# Autodesk Inventor assembly: ActiveClimb-ver2-1111-2020
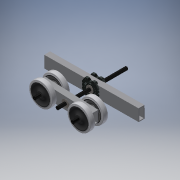
[picture p0: Inventor's stored thumbnail of the model, 180x180]
Saved by Autodesk Inventor 2018 (Build 220112000, 112)
## iProperties
Created: 2020-01-27
Part Number: ActiveClimb-ver2-1111-2020
Document SubType Name: Assembly
Designer: JMHal
Author: JMHal
## Documents named in this file (10)
- G:\PHRC Design Team\GrabCAD\Power Hawks CAD\2020 Infinite Recharge\Active Climb\Assemblies\ActiveClimb-ver2-1111-2020.iam
- G:\PHRC Design Team\GrabCAD\Power Hawks CAD\2020 Infinite Recharge\Active Climb\Parts\AluminumBar-1111-2020.ipt
- G:\PHRC Design Team\GrabCAD\Power Hawks CAD\Resources\VEXpro Resources\Bearings\0.5inHexFlangedBearing(1.125inx0.313in)-1111-2016.ipt
- F:\GrabCad\Resources\VEXpro Resources\Shafts\0.5inThunderHexShaft(8)-1111-2016.ipt
- G:\PHRC Design Team\GrabCAD\Power Hawks CAD\Resources\VEXpro Resources\Wheels\4 inch\4inColsonPerformaWheel-1111-2017.ipt
- G:\PHRC Design Team\GrabCAD\Power Hawks CAD\2020 Infinite Recharge\Active Climb\Parts\2x1 16in Aluminum-ver1-1111-2020.ipt
- G:\PHRC Design Team\GrabCAD\Power Hawks CAD\Resources\VEXpro Resources\Versa Motion\VersaBlockKit-1111-2016.ipt
- G:\PHRC Design Team\GrabCAD\Power Hawks CAD\2020 Infinite Recharge\Active Climb\Parts\12in Hex Shaft-ver1-1111-2020.iam
- G:\PHRC Design Team\GrabCAD\Power Hawks CAD\Resources\VEXpro Resources\Shafts\0.5inThunderHexShaft(8in(modified))-1111-2016.ipt
- G:\PHRC Design Team\GrabCAD\Power Hawks CAD\Resources\VEXpro Resources\Shafts\0.5inThunderHexShaft(5in(modified))-1111-2016.ipt
## Components (22 placed, 9 different names)
1. AluminumBar-1111-2020:1 — Cylindrical:1, Mate:1, Cylindrical:2, Mate:2, Cylindrical:3, Mate:3, Cylindrical:4, Mate:4, Cylindrical:5, Mate:5, Cylindrical:6, Mate:6
2. 0.5inThunderHexShaft(8)-1111-2016:1 — Cylindrical:16, Cylindrical:17, Flush:1, Cylindrical:21
3. 0.5inThunderHexShaft(8)-1111-2016:3 — Cylindrical:19, Flush:3, Cylindrical:20, Cylindrical:22
4. 4inColsonPerformaWheel-1111-2017:1 — Cylindrical:16, Mate:7, Cylindrical:30
5. 4inColsonPerformaWheel-1111-2017:2 — Cylindrical:20, Mate:8, Cylindrical:32
6. 4inColsonPerformaWheel-1111-2017:3 — Cylindrical:21, Mate:9, Cylindrical:34
7. 4inColsonPerformaWheel-1111-2017:4 — Cylindrical:22, Mate:10, Cylindrical:33
8. 2x1 16in Aluminum-ver1-1111-2020:1 — Mate:11, Mate:12, Angle:2, Mate:13, Mate:14, Angle:3
9. VersaBlockKit-1111-2016:1 — Mate:11, Mate:12, Angle:2, Cylindrical:24, Mate:15
10. VersaBlockKit-1111-2016:2 — Mate:13, Mate:14, Angle:3, Cylindrical:25, Mate:16
11. 0.5inHexFlangedBearing(1.125inx0.313in)-1111-2016:7 — Cylindrical:24, Mate:15, Cylindrical:27, Cylindrical:35, Flush:7, Mate:17
12. 0.5inHexFlangedBearing(1.125inx0.313in)-1111-2016:8 — Cylindrical:25, Mate:16
13. 12in Hex Shaft-ver1-1111-2020:1 [sub-assembly] — Cylindrical:26, Cylindrical:27
14. 0.5inThunderHexShaft(5in(modified))-1111-2016:1 — Cylindrical:29, Flush:5, Cylindrical:30, Cylindrical:34
15. 0.5inThunderHexShaft(5in(modified))-1111-2016:2 — Cylindrical:31, Flush:6, Cylindrical:32, Cylindrical:33
16. 0.5inThunderHexShaft(8in(modified))-1111-2016:2 — Cylindrical:35, Flush:7, Cylindrical:36
17. 0.5inHexFlangedBearing(1.125inx0.313in)-1111-2016:2 — Cylindrical:2, Mate:2, Cylindrical:26, Cylindrical:36
18. 0.5inHexFlangedBearing(1.125inx0.313in)-1111-2016:1 — Cylindrical:1, Mate:1, Cylindrical:17, Flush:1, Mate:7, Cylindrical:29, Flush:5
19. 0.5inHexFlangedBearing(1.125inx0.313in)-1111-2016:3 — Cylindrical:3, Mate:3, Cylindrical:19, Flush:3, Mate:8, Cylindrical:31, Flush:6
20. 0.5inHexFlangedBearing(1.125inx0.313in)-1111-2016:4 — Cylindrical:4, Mate:4, Mate:10
21. 0.5inHexFlangedBearing(1.125inx0.313in)-1111-2016:5 — Cylindrical:5, Mate:5, Mate:17
22. 0.5inHexFlangedBearing(1.125inx0.313in)-1111-2016:6 — Cylindrical:6, Mate:6, Mate:9
## Relationships (48: CylindricalJoint 24, Mate 17, Flush 5, Angle 2)
- Cylindrical:1: AluminumBar-1111-2020:1 ↔ 0.5inHexFlangedBearing(1.125inx0.313in)-1111-2016:1
- Mate:1: AluminumBar-1111-2020:1 ↔ 0.5inHexFlangedBearing(1.125inx0.313in)-1111-2016:1
- Cylindrical:2: AluminumBar-1111-2020:1 ↔ 0.5inHexFlangedBearing(1.125inx0.313in)-1111-2016:2
- Mate:2: AluminumBar-1111-2020:1 ↔ 0.5inHexFlangedBearing(1.125inx0.313in)-1111-2016:2
- Cylindrical:3: AluminumBar-1111-2020:1 ↔ 0.5inHexFlangedBearing(1.125inx0.313in)-1111-2016:3
- Mate:3: AluminumBar-1111-2020:1 ↔ 0.5inHexFlangedBearing(1.125inx0.313in)-1111-2016:3
- Cylindrical:4: AluminumBar-1111-2020:1 ↔ 0.5inHexFlangedBearing(1.125inx0.313in)-1111-2016:4
- Mate:4: AluminumBar-1111-2020:1 ↔ 0.5inHexFlangedBearing(1.125inx0.313in)-1111-2016:4
- Cylindrical:5: AluminumBar-1111-2020:1 ↔ 0.5inHexFlangedBearing(1.125inx0.313in)-1111-2016:5
- Mate:5: AluminumBar-1111-2020:1 ↔ 0.5inHexFlangedBearing(1.125inx0.313in)-1111-2016:5
- Cylindrical:6: AluminumBar-1111-2020:1 ↔ 0.5inHexFlangedBearing(1.125inx0.313in)-1111-2016:6
- Mate:6: AluminumBar-1111-2020:1 ↔ 0.5inHexFlangedBearing(1.125inx0.313in)-1111-2016:6
- Cylindrical:16: 0.5inThunderHexShaft(8)-1111-2016:1 ↔ 4inColsonPerformaWheel-1111-2017:1
- Cylindrical:17: 0.5inThunderHexShaft(8)-1111-2016:1 ↔ 0.5inHexFlangedBearing(1.125inx0.313in)-1111-2016:1
- Flush:1 (-50.8 mm): 0.5inThunderHexShaft(8)-1111-2016:1 ↔ 0.5inHexFlangedBearing(1.125inx0.313in)-1111-2016:1
- Cylindrical:19: 0.5inThunderHexShaft(8)-1111-2016:3 ↔ 0.5inHexFlangedBearing(1.125inx0.313in)-1111-2016:3
- Flush:3 (-50.8 mm): 0.5inThunderHexShaft(8)-1111-2016:3 ↔ 0.5inHexFlangedBearing(1.125inx0.313in)-1111-2016:3
- Mate:7: 4inColsonPerformaWheel-1111-2017:1 ↔ 0.5inHexFlangedBearing(1.125inx0.313in)-1111-2016:1
- Cylindrical:20: 0.5inThunderHexShaft(8)-1111-2016:3 ↔ 4inColsonPerformaWheel-1111-2017:2
- Mate:8: 4inColsonPerformaWheel-1111-2017:2 ↔ 0.5inHexFlangedBearing(1.125inx0.313in)-1111-2016:3
- Cylindrical:21: 0.5inThunderHexShaft(8)-1111-2016:1 ↔ 4inColsonPerformaWheel-1111-2017:3
- Mate:9: 4inColsonPerformaWheel-1111-2017:3 ↔ 0.5inHexFlangedBearing(1.125inx0.313in)-1111-2016:6
- Cylindrical:22: 0.5inThunderHexShaft(8)-1111-2016:3 ↔ 4inColsonPerformaWheel-1111-2017:4
- Mate:10: 4inColsonPerformaWheel-1111-2017:4 ↔ 0.5inHexFlangedBearing(1.125inx0.313in)-1111-2016:4
- Mate:11: 2x1 16in Aluminum-ver1-1111-2020:1 ↔ VersaBlockKit-1111-2016:1
- Mate:12: 2x1 16in Aluminum-ver1-1111-2020:1 ↔ VersaBlockKit-1111-2016:1
- Angle:2 (0 deg): 2x1 16in Aluminum-ver1-1111-2020:1 ↔ VersaBlockKit-1111-2016:1
- Mate:13: 2x1 16in Aluminum-ver1-1111-2020:1 ↔ VersaBlockKit-1111-2016:2
- Mate:14: 2x1 16in Aluminum-ver1-1111-2020:1 ↔ VersaBlockKit-1111-2016:2
- Angle:3 (0 deg): 2x1 16in Aluminum-ver1-1111-2020:1 ↔ VersaBlockKit-1111-2016:2
- Cylindrical:24: VersaBlockKit-1111-2016:1 ↔ 0.5inHexFlangedBearing(1.125inx0.313in)-1111-2016:7
- Mate:15: VersaBlockKit-1111-2016:1 ↔ 0.5inHexFlangedBearing(1.125inx0.313in)-1111-2016:7
- Cylindrical:25: VersaBlockKit-1111-2016:2 ↔ 0.5inHexFlangedBearing(1.125inx0.313in)-1111-2016:8
- Mate:16: VersaBlockKit-1111-2016:2 ↔ 0.5inHexFlangedBearing(1.125inx0.313in)-1111-2016:8
- Cylindrical:26: 12in Hex Shaft-ver1-1111-2020:1 ↔ 0.5inHexFlangedBearing(1.125inx0.313in)-1111-2016:2
- Cylindrical:27: 0.5inHexFlangedBearing(1.125inx0.313in)-1111-2016:7 ↔ 12in Hex Shaft-ver1-1111-2020:1
- Cylindrical:29: 0.5inThunderHexShaft(5in(modified))-1111-2016:1 ↔ 0.5inHexFlangedBearing(1.125inx0.313in)-1111-2016:1
- Flush:5 (-50.8 mm): 0.5inThunderHexShaft(5in(modified))-1111-2016:1 ↔ 0.5inHexFlangedBearing(1.125inx0.313in)-1111-2016:1
- Cylindrical:30: 4inColsonPerformaWheel-1111-2017:1 ↔ 0.5inThunderHexShaft(5in(modified))-1111-2016:1
- Cylindrical:31: 0.5inThunderHexShaft(5in(modified))-1111-2016:2 ↔ 0.5inHexFlangedBearing(1.125inx0.313in)-1111-2016:3
- Flush:6 (-50.8 mm): 0.5inThunderHexShaft(5in(modified))-1111-2016:2 ↔ 0.5inHexFlangedBearing(1.125inx0.313in)-1111-2016:3
- Cylindrical:32: 4inColsonPerformaWheel-1111-2017:2 ↔ 0.5inThunderHexShaft(5in(modified))-1111-2016:2
- Cylindrical:33: 4inColsonPerformaWheel-1111-2017:4 ↔ 0.5inThunderHexShaft(5in(modified))-1111-2016:2
- Cylindrical:34: 4inColsonPerformaWheel-1111-2017:3 ↔ 0.5inThunderHexShaft(5in(modified))-1111-2016:1
- Cylindrical:35: 0.5inHexFlangedBearing(1.125inx0.313in)-1111-2016:7 ↔ 0.5inThunderHexShaft(8in(modified))-1111-2016:2
- Flush:7 (-139.7 mm): 0.5inHexFlangedBearing(1.125inx0.313in)-1111-2016:7 ↔ 0.5inThunderHexShaft(8in(modified))-1111-2016:2
- Cylindrical:36: 0.5inThunderHexShaft(8in(modified))-1111-2016:2 ↔ 0.5inHexFlangedBearing(1.125inx0.313in)-1111-2016:2
- Mate:17 (-76.2 mm): 0.5inHexFlangedBearing(1.125inx0.313in)-1111-2016:7 ↔ 0.5inHexFlangedBearing(1.125inx0.313in)-1111-2016:5
